# Autodesk Inventor assembly: шестерни изменяемая траектория
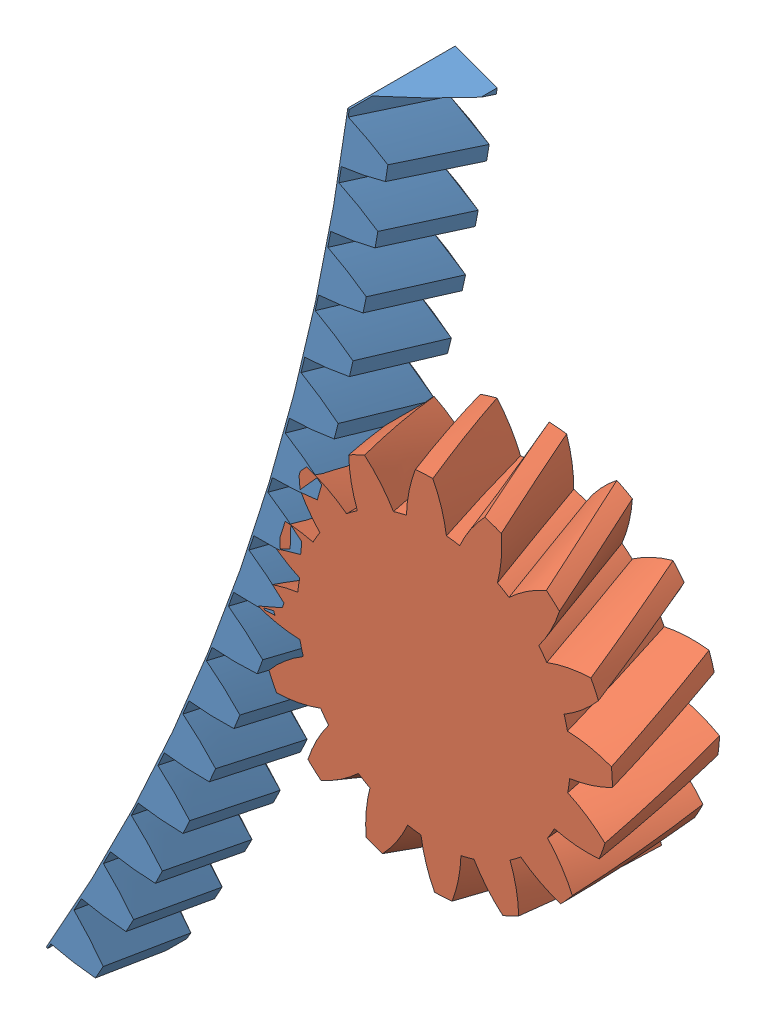
[picture p0: shaded view drawn from the shape stored in the file]
Saved by Autodesk Inventor 2026.2 (Build 302298000, 298)
## iProperties
Created: 2025-12-06
Part Number: шестерни изменяемая траектория
Document SubType Name: Assembly
Designer: Phantom
Author: Phantom
## Documents named in this file (4)
- C:\Users\Phantom\Desktop\Phantom16950\шестерни изменяемая траектория.iam
- C:\Users\Phantom\Desktop\Phantom16950\шестерни изменяемая траектория\Мастер проектирования\Цилиндрическое зубчатое зацепление2.iam
- C:\Users\Phantom\Desktop\Phantom16950\пол шестерни для траектории.ipt
- C:\Users\Phantom\Desktop\Phantom16950\пол шестерни мал для траектории.ipt
## Components (3 placed, 3 different names)
1. Цилиндрическое зубчатое зацепление:2 [sub-assembly]
2. Цилиндрическое зубчатое зацепление1:1 — Заподлицо:1, ЗубчПер:1, Совмещение:10
3. Цилиндрическое зубчатое зацепление2:1 — Заподлицо:1, ЗубчПер:1, Совмещение:10
## Relationships (3: Flush 1, RelateRotation 1, Mate 1)
- Заподлицо:1 [Flush]: Цилиндрическое зубчатое зацепление1:1 ↔ Цилиндрическое зубчатое зацепление2:1
- ЗубчПер:1 [RelateRotation] (0.0667 ul): Цилиндрическое зубчатое зацепление1:1 ↔ Цилиндрическое зубчатое зацепление2:1
- Совмещение:10 [Mate] (239 mm): Цилиндрическое зубчатое зацепление1:1 ↔ Цилиндрическое зубчатое зацепление2:1
